# Autodesk Inventor assembly: Assembly1
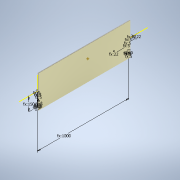
[picture p0: Inventor's stored thumbnail of the model, 180x180]
Saved by Autodesk Inventor 2020 (Build 240168000, 168)
## iProperties
Created: 2021-01-27
Part Number: Assembly1
Document SubType Name: Assembly
Designer: abij996
Author: abij996
## Documents named in this file (4)
- \\files.auckland.ac.nz\myhome\Documents\GitHub\2020-srw-rc-car\CoilDesign\CAD Track\Assembly1.iam
- \\files.auckland.ac.nz\myhome\Documents\GitHub\2020-srw-rc-car\CoilDesign\CAD Track\Wire Cad Model\primary_coil_0R2.ipt
- \\files.auckland.ac.nz\myhome\Documents\GitHub\2020-srw-rc-car\CoilDesign\CAD Track\Ferrite Layer\2 sections\ferrite_section.ipt
- \\files.auckland.ac.nz\myhome\Documents\GitHub\2020-srw-rc-car\CoilDesign\CAD Track\Top Layer\TopCoverLayer.ipt
## Components (8 placed, 3 different names)
1. ferrite_section:1 — Mate:1, Flush:1, Mate:2, Flush:2, Flush:3
2. ferrite_section:2 — Mate:1, Flush:1, Mate:3, Flush:4, Flush:5
3. TopCoverLayer:1 — Flush:4, Flush:5, Mate:6, Flush:9
4. TopCoverLayer:2 — Mate:4, Flush:6, Flush:7, Flush:8
5. TopCoverLayer:3 — Mate:5, Flush:8
6. TopCoverLayer:4 — Mate:6, Flush:9
7. primary_coil_0R2:1 — Mate:2, Flush:2, Flush:3, Mate:3, Mate:4, Flush:6, Flush:7, Mate:5
8. primary_coil_0R2:2
## Component patterns: (2 elements, first: primary_coil_0R2:1)
## Relationships (15: Flush 9, Mate 6)
- Mate:1: ferrite_section:1 ↔ ferrite_section:2
- Flush:1: ferrite_section:1 ↔ ferrite_section:2
- Mate:2: ferrite_section:1 ↔ primary_coil_0R2:1
- Flush:2: ferrite_section:1 ↔ primary_coil_0R2:1
- Flush:3: ferrite_section:1 ↔ primary_coil_0R2:1
- Mate:3: ferrite_section:2 ↔ primary_coil_0R2:1
- Flush:4: ferrite_section:2 ↔ TopCoverLayer:1
- Flush:5: ferrite_section:2 ↔ TopCoverLayer:1
- Mate:4: TopCoverLayer:2 ↔ primary_coil_0R2:1
- Flush:6: TopCoverLayer:2 ↔ primary_coil_0R2:1
- Flush:7: TopCoverLayer:2 ↔ primary_coil_0R2:1
- Mate:5: TopCoverLayer:3 ↔ primary_coil_0R2:1
- Flush:8: TopCoverLayer:2 ↔ TopCoverLayer:3
- Mate:6: TopCoverLayer:1 ↔ TopCoverLayer:4
- Flush:9: TopCoverLayer:1 ↔ TopCoverLayer:4
